# Autodesk Inventor assembly: CLB_051_TorsionSpringSpacerAssembly
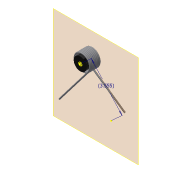
[picture p0: Inventor's stored thumbnail of the model, 180x180]
Saved by Autodesk Inventor 2018 (Build 220112000, 112)
## iProperties
Created: 2020-02-14
Part Number: CLB_051_TorsionSpringSpacerAssembly
Document SubType Name: Assembly
Designer: 22perngrac
Author: 22perngrac
## Documents named in this file (3)
- C:\Users\Myers.000\Documents\GrabCAD\Infinite Recharge 2020\Build season\CLB_051_TorsionSpringSpacerAssembly.iam
- C:\Users\Myers.000\Documents\GrabCAD\Infinite Recharge 2020\Build season\CLB_045_TorsionSpring_MM_9271K129.ipt
- C:\Users\Myers.000\Documents\GrabCAD\Infinite Recharge 2020\Build season\CLB_047_SpringSpacer.ipt
## Components (2 placed, 2 different names)
1. CLB_045_TorsionSpring_MM_9271K129:1
2. CLB_047_SpringSpacer:1 — Mate:1
## Relationships (2: Flush 1, Mate 1)
- Flush:1 (-11.3157 mm)
- Mate:1: CLB_047_SpringSpacer:1
